# Autodesk Inventor assembly: Link1
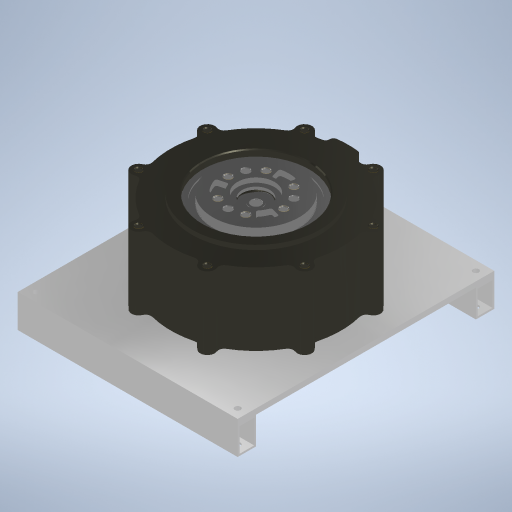
[picture p0: Inventor's stored thumbnail of the model, 512x512]
Saved by Autodesk Inventor 2024 (Build 280153000, 153)
## iProperties
Created: 2024-12-13
Part Number: Link1
Document SubType Name: Assembly
Designer: hirek
Author: hirek
## Documents named in this file (4)
- E:\Documents\Inventor\CanAloha\Link1.iam
- E:\Documents\Inventor\CanAloha\myperts\base_plate2.ipt
- E:\Documents\Inventor\CanAloha\official\robStride03\Robstride03.iam
- E:\Documents\Inventor\CanAloha\myperts\base_pipe1.ipt
## Components (4 placed, 3 different names)
1. base_plate2:1 — 回転:1, 回転:2, 回転:3, 回転:4, 回転:5, 回転:6
2. Robstride03:1 [sub-assembly] — 回転:1, 回転:2
3. base_pipe1:1 — 回転:3, 回転:4
4. base_pipe1:2 — 回転:5, 回転:6
## Relationships (6: RevoluteJoint 6)
- 回転:1 [RevoluteJoint]: base_plate2:1 ↔ Robstride03:1
- 回転:2 [RevoluteJoint]: base_plate2:1 ↔ Robstride03:1
- 回転:3 [RevoluteJoint]: base_plate2:1 ↔ base_pipe1:1
- 回転:4 [RevoluteJoint]: base_plate2:1 ↔ base_pipe1:1
- 回転:5 [RevoluteJoint]: base_plate2:1 ↔ base_pipe1:2
- 回転:6 [RevoluteJoint]: base_plate2:1 ↔ base_pipe1:2
